# Autodesk Inventor assembly: MainAssy_MIR
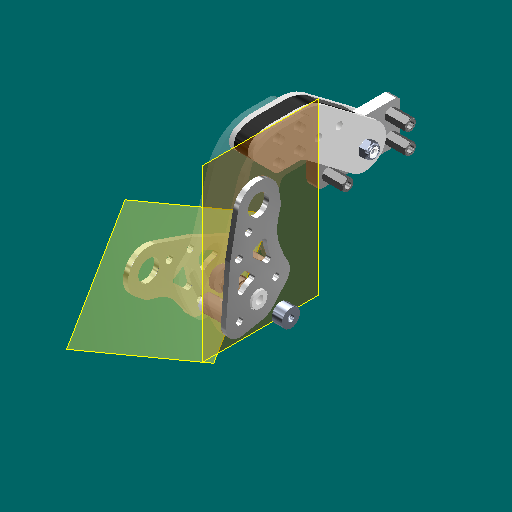
[picture p0: Inventor's stored thumbnail of the model, 512x512]
Saved by Autodesk Inventor 2023.1 (Build 271208000, 208)
## iProperties
Created: 2022-11-06
Part Number: MainAssy_MIR
Document SubType Name: Assembly
Designer: Zac Hah
Mass: 4700.42 g
Surface Area: 13150.1 cm^2
Volume: 2878.83 cm^3
Density: 1.63275 g/cm^3
Author: zac-h
## Documents named in this file (20)
- C:\Users\zac-h\Documents\CAD\spin-up-18_1\IntakeSide_MIR.iam
- IntakeSide_MIR.iam
- C:\Users\zac-h\Documents\CAD\spin-up-18_1\IntakeShoulder_MIR.ipt
- C:\Users\zac-h\Documents\CAD\VEX-CAD-Inventor-1.3.0\VEX-CAD-Inventor-1.3.0\Structure\Standoff\Standoff .50.ipt
- C:\Users\zac-h\Documents\CAD\VEX-CAD-Inventor-1.3.0\VEX-CAD-Inventor-1.3.0\Structure\Hardware\Nut Nylock.ipt
- C:\Users\zac-h\Documents\CAD\VEX-CAD-Inventor-1.3.0\VEX-CAD-Inventor-1.3.0\Motion\Spacers\Washer Teflon\TWasher .375 OD x .04000.ipt
- C:\Users\zac-h\Documents\CAD\VEX-CAD-Inventor-1.3.0\VEX-CAD-Inventor-1.3.0\Structure\Hardware\Screw Steel - Star\SScrew Star Smooth .500.ipt
- C:\Users\Zac Hah\Documents\GitHub\spin-up-cad\VEX-CAD-Inventor-1.3.0\VEX-CAD-Inventor-1.3.0\Structure\Hardware\Screw Steel - Star.ipt
- C:\Users\zac-h\Documents\CAD\spin-up-18_1\IntakeAftArm_MIR.ipt
- C:\Users\zac-h\Documents\CAD\spin-up-18_1\IntakeForearm_MIR.ipt
- C:\Users\zac-h\Documents\CAD\spin-up-18_1\IntakeBearingBlock_MIR.ipt
- C:\Users\zac-h\Documents\CAD\spin-up-18_1\vexbearing_MIR.ipt
- C:\Users\zac-h\Documents\CAD\spin-up-18_1\IntakeBearingSpacer_MIR.ipt
- C:\Users\zac-h\Documents\CAD\guardSwerve5\100spacer_MIR.ipt
- C:\Users\zac-h\Documents\CAD\VEX-CAD-Inventor-1.3.0\VEX-CAD-Inventor-1.3.0\Motion\Wheels\Flex Wheels\2.000 Flex Wheel\2.000 30A .500.ipt
- C:\Users\Zac Hah\Documents\GitHub\spin-up-cad\VEX-CAD-Inventor-1.3.0\VEX-CAD-Inventor-1.3.0\Motion\Wheels\Flex Wheels\2.000 Flex Wheel.ipt
- C:\Users\zac-h\Documents\CAD\VEX-CAD-Inventor-1.3.0\VEX-CAD-Inventor-1.3.0\Motion\Shaft Collar without Set Screw.ipt
- C:\Users\zac-h\Documents\CAD\guardSwerve5\IntakeArmSpacingBlock_MIR.ipt
- C:\Users\zac-h\Documents\CAD\VEX-CAD-Inventor-1.3.0\VEX-CAD-Inventor-1.3.0\Structure\Standoff.ipt
- C:\Users\zac-h\Documents\CAD\VEX-CAD-Inventor-1.3.0\VEX-CAD-Inventor-1.3.0\Motion\Spacers\Washer Teflon.ipt
## Components (27 placed, 14 different names)
1. IntakeShoulder_MIR:1 — Insert:35, Insert:34, Insert:39, Insert:38, Insert:37, Insert:40
2. Standoff .50:1
3. Standoff .50:2 — Insert:35
4. Standoff .50:3
5. Nut Nylock:1 — Insert:42
6. TWasher .375 OD x .04000:1 — Insert:34, Flush:1
7. SScrew Star Smooth .500:1 — Insert:39
8. SScrew Star Smooth .500:2 — Insert:38
9. SScrew Star Smooth .500:3 — Insert:37
10. TWasher .375 OD x .04000:2 — Insert:40, Insert:41
11. IntakeAftArm_MIR:1 — Flush:1, Insert:43
12. IntakeAftArm_MIR:2 — Insert:42, Insert:41, Flush:2, Flush:7
13. IntakeForearm_MIR:1 — Flush:2, Flush:4, Flush:3
14. IntakeForearm_MIR:2 — Insert:43, Insert:45, Insert:44, Insert:52, Flush:5, Insert:49
15. IntakeBearingBlock_MIR:1 — Flush:4, Flush:3, Insert:46
16. IntakeBearingBlock_MIR:2 — Insert:45, Insert:44, Insert:47
17. vexbearing_MIR:1 — Insert:46, Flush:6, Insert:53
18. vexbearing_MIR:2 — Insert:47
19. IntakeBearingSpacer_MIR:1 — Insert:52, Flush:5
20. IntakeBearingSpacer_MIR:2 — Insert:49
21. 100spacer_MIR:1 — Flush:6, Insert:51
22. 2.000 30A .500:1 — Insert:51, Insert:56
23. 100spacer_MIR:2 — Insert:53, Insert:54
24. Shaft Collar without Set Screw:1 — Insert:54, Insert:55
25. 100spacer_MIR:3 — Insert:55
26. Shaft Collar without Set Screw:2 — Insert:56
27. IntakeArmSpacingBlock_MIR:1 — Flush:7
## Relationships (27: Insert 20, Mate 7)
- Insert:35: IntakeShoulder_MIR:1 ↔ Standoff .50:2
- Insert:34: IntakeShoulder_MIR:1 ↔ TWasher .375 OD x .04000:1
- Insert:39: IntakeShoulder_MIR:1 ↔ SScrew Star Smooth .500:1
- Insert:38: IntakeShoulder_MIR:1 ↔ SScrew Star Smooth .500:2
- Insert:37: IntakeShoulder_MIR:1 ↔ SScrew Star Smooth .500:3
- Insert:40: IntakeShoulder_MIR:1 ↔ TWasher .375 OD x .04000:2
- Flush:1 [Mate]: TWasher .375 OD x .04000:1 ↔ IntakeAftArm_MIR:1
- Insert:42: Nut Nylock:1 ↔ IntakeAftArm_MIR:2
- Insert:41: TWasher .375 OD x .04000:2 ↔ IntakeAftArm_MIR:2
- Flush:2 [Mate]: IntakeAftArm_MIR:2 ↔ IntakeForearm_MIR:1
- Insert:43: IntakeAftArm_MIR:1 ↔ IntakeForearm_MIR:2
- Flush:4 [Mate]: IntakeForearm_MIR:1 ↔ IntakeBearingBlock_MIR:1
- Flush:3 [Mate]: IntakeForearm_MIR:1 ↔ IntakeBearingBlock_MIR:1
- Insert:45: IntakeForearm_MIR:2 ↔ IntakeBearingBlock_MIR:2
- Insert:44: IntakeForearm_MIR:2 ↔ IntakeBearingBlock_MIR:2
- Insert:46: IntakeBearingBlock_MIR:1 ↔ vexbearing_MIR:1
- Insert:47: IntakeBearingBlock_MIR:2 ↔ vexbearing_MIR:2
- Insert:52: IntakeForearm_MIR:2 ↔ IntakeBearingSpacer_MIR:1
- Flush:5 [Mate]: IntakeForearm_MIR:2 ↔ IntakeBearingSpacer_MIR:1
- Insert:49: IntakeForearm_MIR:2 ↔ IntakeBearingSpacer_MIR:2
- Flush:6 [Mate]: vexbearing_MIR:1 ↔ 100spacer_MIR:1
- Insert:51: 100spacer_MIR:1 ↔ 2.000 30A .500:1
- Insert:53: vexbearing_MIR:1 ↔ 100spacer_MIR:2
- Insert:54: 100spacer_MIR:2 ↔ Shaft Collar without Set Screw:1
- Insert:55: Shaft Collar without Set Screw:1 ↔ 100spacer_MIR:3
- Insert:56: 2.000 30A .500:1 ↔ Shaft Collar without Set Screw:2
- Flush:7 [Mate]: IntakeAftArm_MIR:2 ↔ IntakeArmSpacingBlock_MIR:1
